# Autodesk Inventor assembly: Holder
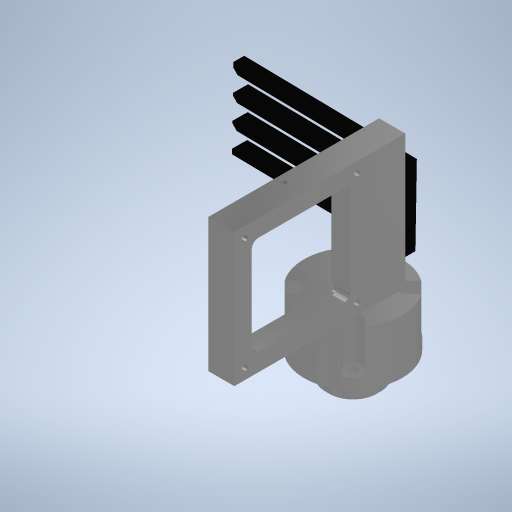
[picture p0: Inventor's stored thumbnail of the model, 512x512]
Saved by Autodesk Inventor 2023 (Build 270158000, 158)
## iProperties
Created: 2021-10-06
Part Number: Holder
Document SubType Name: Assembly
Designer: Timo
Author: Timo
## Documents named in this file (5)
- C:\Users\Timo\Documents\Inventor\Models\Setups\Laserinterferenz\SampleHolder\Sample_Mirror_Holder\Sample_Mirror_Holder.iam
- C:\Users\Timo\Documents\Inventor\Models\Setups\Laserinterferenz\SampleHolder\Sample_Mirror_Holder\MirrorHolder.ipt
- C:\Users\Timo\Documents\Inventor\Models\Setups\Laserinterferenz\SampleHolder\Sample_Mirror_Holder\SampleMountFingers.ipt
- C:\Users\Timo\Documents\Inventor\Models\Setups\Laserinterferenz\SampleHolder\Sample_Mirror_Holder\StageConnection.ipt
- C:\Users\Timo\Documents\Inventor\Content Center Files\R2022\en-US\DIN 912\DIN 912 - M3 x 0,5 x 12 x 10,75.ipt
## Components (8 placed, 4 different names)
1. MirrorHolder:1 — Mate:1, Mate:3, Rigid:1, Rigid:2
2. SampleMountFingers:1 — Flush:1, Rigid:2, Rotational:1, Rotational:2, Rotational:3
3. StageConnection:1 — Mate:1, Mate:4, Rigid:1, Rotational:4, Rotational:5
4. DIN 912 - replaced by DIN EN ISO 4762 M3 x 12:1 — Rotational:4
5. DIN 912 - replaced by DIN EN ISO 4762 M3 x 12:2 — Rotational:1
6. DIN 912 - replaced by DIN EN ISO 4762 M3 x 12:3 — Rotational:2
7. DIN 912 - replaced by DIN EN ISO 4762 M3 x 12:4 — Rotational:5
8. DIN 912 - replaced by DIN EN ISO 4762 M3 x 12:5 — Rotational:3
## Relationships (12: RevoluteJoint 5, Mate 4, WeldJoint 2, Flush 1)
- Mate:1: MirrorHolder:1 ↔ StageConnection:1
- Flush:1 (12 mm): SampleMountFingers:1
- Mate:2
- Mate:3: MirrorHolder:1
- Mate:4: StageConnection:1
- Rigid:1 [WeldJoint]: MirrorHolder:1 ↔ StageConnection:1
- Rigid:2 [WeldJoint]: MirrorHolder:1 ↔ SampleMountFingers:1
- Rotational:1 [RevoluteJoint]: SampleMountFingers:1 ↔ DIN 912 - replaced by DIN EN ISO 4762 M3 x 12:2
- Rotational:2 [RevoluteJoint]: SampleMountFingers:1 ↔ DIN 912 - replaced by DIN EN ISO 4762 M3 x 12:3
- Rotational:3 [RevoluteJoint]: SampleMountFingers:1 ↔ DIN 912 - replaced by DIN EN ISO 4762 M3 x 12:5
- Rotational:4 [RevoluteJoint]: StageConnection:1 ↔ DIN 912 - replaced by DIN EN ISO 4762 M3 x 12:1
- Rotational:5 [RevoluteJoint]: StageConnection:1 ↔ DIN 912 - replaced by DIN EN ISO 4762 M3 x 12:4
